# Autodesk Inventor assembly: launcher.mainAssembly2
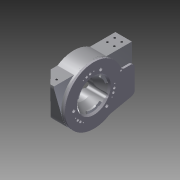
[picture p0: Inventor's stored thumbnail of the model, 180x180]
Saved by Autodesk Inventor 2011 (Build 150239000, 239)
## iProperties
Created: 2011-04-12
Part Number: launcher.mainAssembly2
Document SubType Name: Assembly
Designer: Rob
Author: Rob
## Documents named in this file (6)
- C:\Users\Rob\Dropbox\RockSAT-X 2011 RexSAT\capsule-launcher.design\Launcher\launcher.mainAssembly2.iam
- C:\Users\Rob\Dropbox\RockSAT-X 2011 RexSAT\capsule-launcher.design\Launcher\launcher.housing2.ipt
- C:\Users\Rob\Dropbox\RockSAT-X 2011 RexSAT\capsule-launcher.design\Launcher\3x8x4_bearing.ipt
- C:\Users\Rob\Dropbox\RockSAT-X 2011 RexSAT\capsule-launcher.design\Launcher\launcher.latch.ipt
- C:\Users\Rob\Dropbox\RockSAT-X 2011 RexSAT\capsule-launcher.design\Launcher\launcher.cam.ipt
- C:\Users\Rob\Dropbox\RockSAT-X 2011 RexSAT\capsule-launcher.design\Launcher\launcher.cap2.ipt
## Components (12 placed, 5 different names)
1. launcher.housing2:1 — Mate:1, Mate:2, Mate:3, Mate:4, Mate:5, Mate:6, Mate:7, Mate:8, Mate:9, Mate:10, Mate:11, Mate:12, Mate:13, Mate:14, Mate:15, Mate:16, Mate:18
2. 3x8x4_bearing:1 — Mate:3, Mate:4
3. 3x8x4_bearing:2 — Mate:5, Mate:6
4. 3x8x4_bearing:3 — Mate:1, Mate:2
5. 3x8x4_bearing:4 — Mate:7, Mate:8
6. 3x8x4_bearing:5 — Mate:11, Mate:12
7. 3x8x4_bearing:6 — Mate:9, Mate:10
8. launcher.cam:1 — Mate:15, Mate:16, Mate:17
9. launcher.cap2:1 — Mate:17, Mate:18, Mate:19
10. launcher.latch:1 — Mate:13, Mate:14
11. launcher.latch:2 — Mate:19
12. launcher.latch:3
## Component patterns: (3 elements, first: launcher.latch:1)
## Relationships (19: Mate 19)
- Mate:1: launcher.housing2:1 ↔ 3x8x4_bearing:3
- Mate:2: launcher.housing2:1 ↔ 3x8x4_bearing:3
- Mate:3: launcher.housing2:1 ↔ 3x8x4_bearing:1
- Mate:4: launcher.housing2:1 ↔ 3x8x4_bearing:1
- Mate:5: launcher.housing2:1 ↔ 3x8x4_bearing:2
- Mate:6: launcher.housing2:1 ↔ 3x8x4_bearing:2
- Mate:7: launcher.housing2:1 ↔ 3x8x4_bearing:4
- Mate:8: launcher.housing2:1 ↔ 3x8x4_bearing:4
- Mate:9: launcher.housing2:1 ↔ 3x8x4_bearing:6
- Mate:10: launcher.housing2:1 ↔ 3x8x4_bearing:6
- Mate:11: launcher.housing2:1 ↔ 3x8x4_bearing:5
- Mate:12: launcher.housing2:1 ↔ 3x8x4_bearing:5
- Mate:13: launcher.housing2:1 ↔ launcher.latch:1
- Mate:14: launcher.housing2:1 ↔ launcher.latch:1
- Mate:15: launcher.housing2:1 ↔ launcher.cam:1
- Mate:16: launcher.housing2:1 ↔ launcher.cam:1
- Mate:17: launcher.cam:1 ↔ launcher.cap2:1
- Mate:18: launcher.housing2:1 ↔ launcher.cap2:1
- Mate:19: launcher.cap2:1 ↔ launcher.latch:2
